# Autodesk Inventor assembly: 240628_final
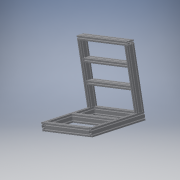
[picture p0: Inventor's stored thumbnail of the model, 180x180]
Saved by Autodesk Inventor 2016 (Build 200138000, 138)
## iProperties
Created: 2024-06-28
Part Number: 240628_final
Material: 일반
Document SubType Name: Assembly
Designer: pc
Author: pc
## Documents named in this file (3)
- D:\CAD_HCH\240628\240628_final.iam
- D:\CAD_HCH\240628\240628_final5(600).ipt
- D:\CAD_HCH\240628\240628_final5(680).ipt
## Components (10 placed, 2 different names)
1. 240628_final5(600):1 — 메이트:1, 플러쉬:1, 플러쉬:2, 메이트:4, 플러쉬:7, 플러쉬:8, 플러쉬:13
2. 240628_final5(680):1 — 메이트:1, 플러쉬:1, 플러쉬:2, 메이트:2, 플러쉬:3, 플러쉬:4
3. 240628_final5(600):2 — 메이트:2, 플러쉬:3, 플러쉬:4, 메이트:3, 플러쉬:5, 플러쉬:6, 메이트:7, 메이트:8, 플러쉬:14
4. 240628_final5(600):3 — 메이트:3, 플러쉬:5, 플러쉬:6, 플러쉬:9, 메이트:5, 플러쉬:10, 메이트:9, 플러쉬:15
5. 240628_final5(600):4 — 메이트:4, 플러쉬:7, 플러쉬:8, 메이트:6, 플러쉬:11, 플러쉬:12
6. 240628_final5(600):5 — 메이트:7, 플러쉬:13
7. 240628_final5(600):6 — 메이트:8, 플러쉬:14
8. 240628_final5(600):7 — 플러쉬:9, 메이트:5, 플러쉬:10
9. 240628_final5(600):8 — 메이트:9, 플러쉬:15
10. 240628_final5(600):9 — 메이트:6, 플러쉬:11, 플러쉬:12
## Relationships (24: Flush 15, Mate 9)
- 메이트:1 [Mate]: 240628_final5(600):1 ↔ 240628_final5(680):1
- 플러쉬:1 [Flush]: 240628_final5(600):1 ↔ 240628_final5(680):1
- 플러쉬:2 [Flush]: 240628_final5(600):1 ↔ 240628_final5(680):1
- 메이트:2 [Mate]: 240628_final5(680):1 ↔ 240628_final5(600):2
- 플러쉬:3 [Flush]: 240628_final5(680):1 ↔ 240628_final5(600):2
- 플러쉬:4 [Flush]: 240628_final5(680):1 ↔ 240628_final5(600):2
- 메이트:3 [Mate]: 240628_final5(600):2 ↔ 240628_final5(600):3
- 플러쉬:5 [Flush]: 240628_final5(600):2 ↔ 240628_final5(600):3
- 플러쉬:6 [Flush]: 240628_final5(600):2 ↔ 240628_final5(600):3
- 메이트:4 [Mate]: 240628_final5(600):1 ↔ 240628_final5(600):4
- 플러쉬:7 [Flush]: 240628_final5(600):1 ↔ 240628_final5(600):4
- 플러쉬:8 [Flush]: 240628_final5(600):1 ↔ 240628_final5(600):4
- 플러쉬:9 [Flush]: 240628_final5(600):3 ↔ 240628_final5(600):7
- 메이트:5 [Mate]: 240628_final5(600):3 ↔ 240628_final5(600):7
- 플러쉬:10 [Flush]: 240628_final5(600):3 ↔ 240628_final5(600):7
- 메이트:6 [Mate]: 240628_final5(600):4 ↔ 240628_final5(600):9
- 플러쉬:11 [Flush]: 240628_final5(600):4 ↔ 240628_final5(600):9
- 플러쉬:12 [Flush]: 240628_final5(600):4 ↔ 240628_final5(600):9
- 메이트:7 [Mate]: 240628_final5(600):2 ↔ 240628_final5(600):5
- 플러쉬:13 [Flush]: 240628_final5(600):1 ↔ 240628_final5(600):5
- 메이트:8 [Mate]: 240628_final5(600):2 ↔ 240628_final5(600):6
- 플러쉬:14 [Flush]: 240628_final5(600):2 ↔ 240628_final5(600):6
- 메이트:9 [Mate]: 240628_final5(600):3 ↔ 240628_final5(600):8
- 플러쉬:15 [Flush]: 240628_final5(600):3 ↔ 240628_final5(600):8
